# Autodesk Inventor assembly: valve_splitter_input
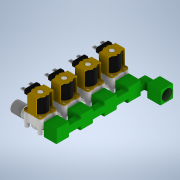
[picture p0: Inventor's stored thumbnail of the model, 180x180]
Saved by Autodesk Inventor 2020 (Build 240168000, 168)
## iProperties
Created: 2020-08-10
Part Number: valve_splitter_input
Document SubType Name: Assembly
Designer: Abbas
Author: Abbas
## Documents named in this file (3)
- C:\Users\LENOVO\Desktop\Graduation Project\Fish Farming Unit\Water Loop Components\valve_splitter_input.iam
- C:\Users\LENOVO\Desktop\Graduation Project\Fish Farming Unit\Water Loop Components\water splitter.ipt
- C:\Users\LENOVO\Desktop\Graduation Project\Fish Farming Unit\Water Loop Components\Solenoid Valve.iam
## Components (5 placed, 2 different names)
1. water splitter:1 — Insert:1, Insert:2, Insert:3, Insert:4
2. Solenoid Valve:1 [sub-assembly] — Insert:1
3. Solenoid Valve:2 [sub-assembly] — Insert:2
4. Solenoid Valve:3 [sub-assembly] — Insert:3
5. Solenoid Valve:4 [sub-assembly] — Insert:4
## Relationships (4: Insert 4)
- Insert:1 (-20 mm): water splitter:1 ↔ Solenoid Valve:1
- Insert:2 (-20 mm): water splitter:1 ↔ Solenoid Valve:2
- Insert:3 (-20 mm): water splitter:1 ↔ Solenoid Valve:3
- Insert:4 (-20 mm): water splitter:1 ↔ Solenoid Valve:4
